# Autodesk Inventor assembly: elbowassembly
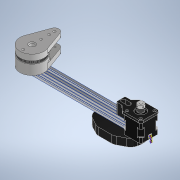
[picture p0: Inventor's stored thumbnail of the model, 180x180]
Saved by Autodesk Inventor 2022 (Build 260153000, 153)
## iProperties
Created: 2022-02-22
Part Number: elbowassembly
Document SubType Name: Assembly
Designer: JK
Author: JK
## Documents named in this file (10)
- C:\Users\JK\Documents\Inventor\ScaraNema\SCARA-3DP\Parts\Elbow\Elbow assembly.iam
- C:\Users\JK\Documents\Inventor\ScaraNema\SCARA-3DP\Parts\Elbow\MOTOR_LONG.ipt
- C:\Users\JK\Documents\Inventor\ScaraNema\SCARA-3DP\Parts\Elbow\RoboDigg GT2 16 pulley.ipt
- C:\Users\JK\Documents\Inventor\ScaraNema\V-Slot 20x20.ipt
- C:\Users\JK\Documents\Inventor\ScaraNema\SCARA-3DP\Parts\Elbow\Elbow pulley.ipt
- C:\Users\JK\Documents\Inventor\ScaraNema\SCARA-3DP\Parts\Elbow\Elbow motor support.ipt
- C:\Users\JK\Documents\Inventor\ScaraNema\SCARA-3DP\Parts\V-Slot 20x20\V-Slot 20x20-250.ipt
- C:\Users\JK\Documents\Inventor\ScaraNema\SCARA-3DP\Parts\Elbow\Bearing support.ipt
- C:\Users\JK\Documents\Inventor\ScaraNema\SCARA-3DP\Parts\Elbow\Platform.ipt
- C:\Users\JK\Documents\Inventor\ScaraNema\SCARA-3DP\Parts\Elbow\Beam support.ipt
## Components (8 placed, 8 different names)
1. MOTOR_LONG:1 — Coincidencia:1, Coincidencia:3, Coincidencia:7, Ángulo:1
2. RoboDigg GT2 16 pulley:1 — Coincidencia:1, Coincidencia:3, Nivelación:3, Coincidencia:6
3. V-Slot 20x20-250:2 — Coincidencia:8, Ángulo:2, Nivelación:4
4. Elbow pulley:1 — Nivelación:3, Coincidencia:4, Coincidencia:5, Coincidencia:10, Coincidencia:11, Coincidencia:12
5. Elbow motor support:1 — Coincidencia:6, Coincidencia:7, Ángulo:1, Coincidencia:9
6. Bearing support:1 — Coincidencia:4, Coincidencia:5
7. Platform:1 — Coincidencia:8, Ángulo:2, Nivelación:4, Coincidencia:9
8. Beam support:1 — Coincidencia:10, Coincidencia:11, Coincidencia:12
## Relationships (18: Mate 12, Flush 4, Angle 2)
- Coincidencia:1 [Mate]: MOTOR_LONG:1 ↔ RoboDigg GT2 16 pulley:1
- [Mate]: MOTOR_LONG:1 ↔ V-Slot 20x20-250:2
- [Flush] (10.75 mm): MOTOR_LONG:1 ↔ V-Slot 20x20-250:2
- [Flush]: MOTOR_LONG:1 ↔ V-Slot 20x20-250:2
- Coincidencia:3 [Mate] (3 mm): MOTOR_LONG:1 ↔ RoboDigg GT2 16 pulley:1
- Nivelación:3 [Flush]: RoboDigg GT2 16 pulley:1 ↔ Elbow pulley:1
- Coincidencia:4 [Mate]: Elbow pulley:1 ↔ Bearing support:1
- Coincidencia:5 [Mate]: Elbow pulley:1 ↔ Bearing support:1
- Coincidencia:6 [Mate]: RoboDigg GT2 16 pulley:1 ↔ Elbow motor support:1
- Coincidencia:7 [Mate]: MOTOR_LONG:1 ↔ Elbow motor support:1
- Ángulo:1 [Angle] (0 deg): MOTOR_LONG:1 ↔ Elbow motor support:1
- Coincidencia:8 [Mate]: V-Slot 20x20-250:2 ↔ Platform:1
- Ángulo:2 [Angle] (180 deg): V-Slot 20x20-250:2 ↔ Platform:1
- Nivelación:4 [Flush]: V-Slot 20x20-250:2 ↔ Platform:1
- Coincidencia:9 [Mate]: Elbow motor support:1 ↔ Platform:1
- Coincidencia:10 [Mate]: Elbow pulley:1 ↔ Beam support:1
- Coincidencia:11 [Mate]: Elbow pulley:1 ↔ Beam support:1
- Coincidencia:12 [Mate]: Elbow pulley:1 ↔ Beam support:1
